# Autodesk Inventor assembly: YAxisIdlerRight
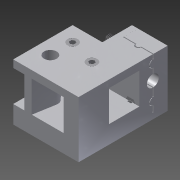
[picture p0: Inventor's stored thumbnail of the model, 180x180]
Saved by Autodesk Inventor 2015 (Build 190159000, 159)
## iProperties
Created: 2014-08-09
Part Number: YAxisIdlerRight
Document SubType Name: Assembly
Designer: Jack
Author: Jack
## Documents named in this file (11)
- C:\Users\t_clevj\ownCloud\CoreXY\InventorModel\YAxis\YAxisIdler\YAxisIdlerRight.iam
- C:\Users\t_clevj\ownCloud\CoreXY\InventorModel\YAxis\YAxisIdler\YAxisIdlerBlockRight.ipt
- C:\Users\t_clevj\ownCloud\CoreXY\InventorModel\YAxis\YAxisIdler\YAxisIdlerCapRight.ipt
- C:\Users\t_clevj\ownCloud\CoreXY\InventorModel\Hardware\Bolts\SHCS\SHCS4\SHCS4x35.ipt
- C:\Users\t_clevj\ownCloud\CoreXY\InventorModel\Hardware\Nuts\Nut4.ipt
- C:\Users\t_clevj\ownCloud\CoreXY\InventorModel\Hardware\Bolts\SHCS\SHCS4\SHCS4x15.ipt
- C:\Users\t_clevj\ownCloud\CoreXY\InventorModel\Hardware\Bolts\SHCS\SHCS5\SHCS5x10.ipt
- C:\Users\t_clevj\ownCloud\CoreXY\InventorModel\Hardware\Bolts\FHS\FHS5\5x10FHS.ipt
- C:\Users\t_clevj\ownCloud\CoreXY\InventorModel\Hardware\Bearing\BearingRadialBall\BearingRadialBallF624zz.ipt
- C:\Users\t_clevj\ownCloud\CoreXY\InventorModel\Hardware\Wahsers\M4Washer.ipt
- C:\Users\t_clevj\ownCloud\CoreXY\InventorModel\YAxis\YAxisIdler\YAxisIdlerBearingSpacer.ipt
## Components (24 placed, 10 different names)
1. YAxisIdlerBlockRight:1 — Flush:3, Mate:3, Mate:2, Flush:2, Flush:1, Mate:1, Mate:7, Mate:4, Mate:6, Mate:5, Angle:2, Mate:10, Mate:11, Angle:1, Mate:14, Mate:12, Mate:22, Mate:21, Flush:4, Mate:20, Mate:35, Mate:37, Mate:38, Mate:39, Mate:40, Mate:41
2. YAxisIdlerCapRight:1 — Flush:2, Flush:1, Mate:1, Mate:18, Mate:16, Mate:19, Mate:17
3. SHCS4x35:1 — Mate:7, Mate:4, Mate:8, Mate:34, Mate:43
4. SHCS4x35:2 — Mate:6, Mate:5, Mate:9, Mate:36, Mate:45
5. Nut4:1 — Angle:2, Mate:10, Mate:8
6. Nut4:2 — Mate:11, Mate:9, Angle:1
7. Nut4:3 — Mate:14
8. Nut4:4 — Mate:12
9. SHCS4x15:1 — Mate:18, Mate:16
10. SHCS4x15:2 — Mate:19, Mate:17
11. SHCS5x10:1 — Mate:22, Mate:21
12. 5x10FHS:1 — Flush:4, Mate:20
13. BearingRadialBallF624zz:1
14. BearingRadialBallF624zz:2
15. M4Washer:1 — Mate:42
16. M4Washer:2 — Mate:34, Mate:35
17. BearingRadialBallF624zz:3
18. BearingRadialBallF624zz:4
19. M4Washer:3 — Mate:37
20. M4Washer:4 — Mate:36, Mate:44
21. SHCS5x10:2 — Mate:38, Mate:41
22. SHCS5x10:3 — Mate:39, Mate:40
23. YAxisIdlerBearingSpacer:1 — Mate:44, Mate:45
24. YAxisIdlerBearingSpacer:2 — Mate:42, Mate:43
## Relationships (50: Mate 43, Flush 5, Angle 2)
- Flush:3: YAxisIdlerBlockRight:1
- Mate:3 [Flush]: YAxisIdlerBlockRight:1
- Mate:2: YAxisIdlerBlockRight:1
- Flush:2: YAxisIdlerBlockRight:1 ↔ YAxisIdlerCapRight:1
- Flush:1: YAxisIdlerBlockRight:1 ↔ YAxisIdlerCapRight:1
- Mate:1: YAxisIdlerBlockRight:1 ↔ YAxisIdlerCapRight:1
- Mate:7: YAxisIdlerBlockRight:1 ↔ SHCS4x35:1
- Mate:4: YAxisIdlerBlockRight:1 ↔ SHCS4x35:1
- Mate:6: YAxisIdlerBlockRight:1 ↔ SHCS4x35:2
- Mate:5: YAxisIdlerBlockRight:1 ↔ SHCS4x35:2
- Angle:2 (0 deg): YAxisIdlerBlockRight:1 ↔ Nut4:1
- Mate:10: YAxisIdlerBlockRight:1 ↔ Nut4:1
- Mate:8: SHCS4x35:1 ↔ Nut4:1
- Mate:11: YAxisIdlerBlockRight:1 ↔ Nut4:2
- Mate:9: SHCS4x35:2 ↔ Nut4:2
- Angle:1 (0 deg): YAxisIdlerBlockRight:1 ↔ Nut4:2
- Mate:14: YAxisIdlerBlockRight:1 ↔ Nut4:3
- Mate:12: YAxisIdlerBlockRight:1 ↔ Nut4:4
- Mate:18: YAxisIdlerCapRight:1 ↔ SHCS4x15:1
- Mate:16: YAxisIdlerCapRight:1 ↔ SHCS4x15:1
- Mate:19: YAxisIdlerCapRight:1 ↔ SHCS4x15:2
- Mate:17: YAxisIdlerCapRight:1 ↔ SHCS4x15:2
- Mate:22: YAxisIdlerBlockRight:1 ↔ SHCS5x10:1
- Mate:21: YAxisIdlerBlockRight:1 ↔ SHCS5x10:1
- Flush:4: YAxisIdlerBlockRight:1 ↔ 5x10FHS:1
- Mate:20: YAxisIdlerBlockRight:1 ↔ 5x10FHS:1
- [Mate]: BearingRadialBallF624zz:1 ↔ BearingRadialBallF624zz:2
- [Mate]: BearingRadialBallF624zz:1 ↔ BearingRadialBallF624zz:2
- [Mate]: BearingRadialBallF624zz:1 ↔ M4Washer:1
- [Mate]: BearingRadialBallF624zz:2 ↔ M4Washer:1
- [Mate]: BearingRadialBallF624zz:1 ↔ M4Washer:2
- [Mate]: BearingRadialBallF624zz:1 ↔ M4Washer:2
- [Mate]: BearingRadialBallF624zz:3 ↔ BearingRadialBallF624zz:4
- [Mate]: BearingRadialBallF624zz:3 ↔ BearingRadialBallF624zz:4
- [Mate]: BearingRadialBallF624zz:3 ↔ M4Washer:3
- [Mate]: BearingRadialBallF624zz:4 ↔ M4Washer:3
- [Mate]: BearingRadialBallF624zz:3 ↔ M4Washer:4
- [Mate]: BearingRadialBallF624zz:3 ↔ M4Washer:4
- Mate:34: SHCS4x35:1 ↔ M4Washer:2
- Mate:35: YAxisIdlerBlockRight:1 ↔ M4Washer:2
- Mate:36: SHCS4x35:2 ↔ M4Washer:4
- Mate:37: YAxisIdlerBlockRight:1 ↔ M4Washer:3
- Mate:38: YAxisIdlerBlockRight:1 ↔ SHCS5x10:2
- Mate:39: YAxisIdlerBlockRight:1 ↔ SHCS5x10:3
- Mate:40: YAxisIdlerBlockRight:1 ↔ SHCS5x10:3
- Mate:41: YAxisIdlerBlockRight:1 ↔ SHCS5x10:2
- Mate:42: M4Washer:1 ↔ YAxisIdlerBearingSpacer:2
- Mate:43: SHCS4x35:1 ↔ YAxisIdlerBearingSpacer:2
- Mate:44: M4Washer:4 ↔ YAxisIdlerBearingSpacer:1
- Mate:45: SHCS4x35:2 ↔ YAxisIdlerBearingSpacer:1
## Named parameters: d63_d160 = 0 mm, d64_d161 = 0 mm, d65_d162 = 0 mm, d66_d163 = 0 mm, d67_d158 = 0 mm, d68_d159 = 0 mm
